# Autodesk Inventor assembly: scrambler_assy1
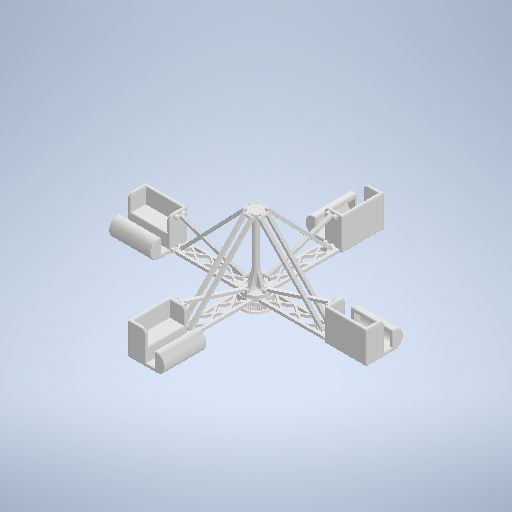
[picture p0: Inventor's stored thumbnail of the model, 512x512]
Saved by Autodesk Inventor 2025.2 (Build 292293000, 293)
## iProperties
Created: 2025-10-10
Part Number: scrambler_assy1
Document SubType Name: Assembly
Designer: pascu
Author: pascu
## Documents named in this file (8)
- C:\Users\pascu\OneDrive\Documents\GitHub\amusement-park\scrambler_assy1.iam
- C:\Users\pascu\OneDrive\Documents\GitHub\amusement-park\scrambler_chariot.ipt
- C:\Users\pascu\OneDrive\Documents\GitHub\amusement-park\scrambler_spider_beam.ipt
- C:\Users\pascu\OneDrive\Documents\GitHub\amusement-park\scrambler_vertical_outer.ipt
- C:\Users\pascu\OneDrive\Documents\GitHub\amusement-park\scrambler_spider_support1.ipt
- C:\Users\pascu\OneDrive\Documents\GitHub\amusement-park\scrambler_vertical_cap.ipt
- C:\Users\pascu\OneDrive\Documents\GitHub\amusement-park\scrambler_spider_support2.ipt
- C:\Users\pascu\OneDrive\Documents\GitHub\amusement-park\spider_gears\Design Accelerator\Spur Gear11.ipt
## Components (23 placed, 7 different names)
1. scrambler_chariot:1 — Mate:1, Angle:1, Flush:1
2. scrambler_spider_beam:1 — Mate:1, Angle:1, Flush:1, Mate:2, Mate:3
3. scrambler_vertical_outer:1 — Mate:2, Mate:3, Mate:8, Mate:9, Mate:10, Mate:11, Mate:12, Mate:13, Mate:16, Mate:17, Mate:22, Mate:23
4. scrambler_chariot:2 — Mate:14, Mate:15
5. scrambler_spider_beam:2 — Mate:8, Mate:9
6. scrambler_chariot:3
7. scrambler_spider_beam:3 — Mate:12, Mate:13, Angle:5, Mate:18, Mate:19, Mate:20, Mate:21
8. scrambler_chariot:4
9. scrambler_spider_beam:4 — Mate:10, Mate:11
10. scrambler_vertical_cap:1 — Mate:16, Mate:17, Angle:5
11. Spur Gear1:1 — Mate:22, Mate:23
12. scrambler_spider_support1:1 — Mate:14, Mate:15
13. scrambler_spider_support1:2
14. scrambler_spider_support1:3
15. scrambler_spider_support1:4
16. scrambler_spider_support2:1 — Mate:18, Mate:19
17. scrambler_spider_support2:2 — Mate:20, Mate:21
18. scrambler_spider_support2:3
19. scrambler_spider_support2:4
20. scrambler_spider_support2:5
21. scrambler_spider_support2:6
22. scrambler_spider_support2:7
23. scrambler_spider_support2:8
## Component patterns: (4 elements, first: scrambler_spider_support1:1), (4 elements, first: scrambler_spider_support2:1 + scrambler_spider_support2:2)
## Relationships (31: Mate 22, Angle 5, Flush 4)
- Mate:1: scrambler_chariot:1 ↔ scrambler_spider_beam:1
- Angle:1 (0 deg): scrambler_chariot:1 ↔ scrambler_spider_beam:1
- Flush:1 (-11.43 mm): scrambler_chariot:1 ↔ scrambler_spider_beam:1
- Mate:2: scrambler_spider_beam:1 ↔ scrambler_vertical_outer:1
- Mate:3: scrambler_spider_beam:1 ↔ scrambler_vertical_outer:1
- [Mate]: scrambler_chariot:2 ↔ scrambler_spider_beam:2
- [Angle] (0 deg): scrambler_chariot:2 ↔ scrambler_spider_beam:2
- [Flush] (-11.43 mm): scrambler_chariot:2 ↔ scrambler_spider_beam:2
- [Mate]: scrambler_chariot:3 ↔ scrambler_spider_beam:3
- [Angle] (0 deg): scrambler_chariot:3 ↔ scrambler_spider_beam:3
- [Flush] (-11.43 mm): scrambler_chariot:3 ↔ scrambler_spider_beam:3
- [Mate]: scrambler_chariot:4 ↔ scrambler_spider_beam:4
- [Angle] (0 deg): scrambler_chariot:4 ↔ scrambler_spider_beam:4
- [Flush] (-11.43 mm): scrambler_chariot:4 ↔ scrambler_spider_beam:4
- Mate:8: scrambler_vertical_outer:1 ↔ scrambler_spider_beam:2
- Mate:9: scrambler_vertical_outer:1 ↔ scrambler_spider_beam:2
- Mate:10: scrambler_vertical_outer:1 ↔ scrambler_spider_beam:4
- Mate:11: scrambler_vertical_outer:1 ↔ scrambler_spider_beam:4
- Mate:12: scrambler_vertical_outer:1 ↔ scrambler_spider_beam:3
- Mate:13: scrambler_vertical_outer:1 ↔ scrambler_spider_beam:3
- Mate:14: scrambler_chariot:2 ↔ scrambler_spider_support1:1
- Mate:15: scrambler_chariot:2 ↔ scrambler_spider_support1:1
- Mate:16: scrambler_vertical_outer:1 ↔ scrambler_vertical_cap:1
- Mate:17: scrambler_vertical_outer:1 ↔ scrambler_vertical_cap:1
- Angle:5 (0 deg): scrambler_spider_beam:3 ↔ scrambler_vertical_cap:1
- Mate:18: scrambler_spider_beam:3 ↔ scrambler_spider_support2:1
- Mate:19: scrambler_spider_beam:3 ↔ scrambler_spider_support2:1
- Mate:20: scrambler_spider_beam:3 ↔ scrambler_spider_support2:2
- Mate:21: scrambler_spider_beam:3 ↔ scrambler_spider_support2:2
- Mate:22: scrambler_vertical_outer:1 ↔ Spur Gear1:1
- Mate:23: scrambler_vertical_outer:1 ↔ Spur Gear1:1
## Named parameters: d7_d1 = 0 mm, d8_d2 = 0 deg, d9_d3 = -11.43 mm, d10_d1 = 0 mm, d11_d2 = 0 deg, d12_d3 = -11.43 mm, d13_d1 = 0 mm, d14_d2 = 0 deg, d15_d3 = -11.43 mm
